# Autodesk Inventor assembly: chaimber
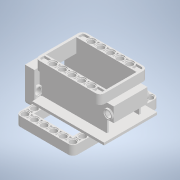
[picture p0: Inventor's stored thumbnail of the model, 180x180]
Saved by Autodesk Inventor 2021 (Build 250183000, 183)
## iProperties
Created: 2024-03-18
Part Number: chaimber
Document SubType Name: Assembly
Designer: 22hamfri
Author: 22hamfri
## Documents named in this file (5)
- C:\Users\22hamfri\Documents\School\Programmering\domino-bil\CAD\chaimber.iam
- C:\Users\22hamfri\Documents\School\Programmering\domino-bil\CAD\chaimber.ipt
- C:\Users\22hamfri\Documents\School\Programmering\domino-bil\CAD\chaimber-adapter.ipt
- C:\Users\22hamfri\Documents\School\Programmering\domino-bil\CAD\vehicle-adapter.ipt
- C:\Users\22hamfri\Documents\School\Programmering\domino-bil\CAD\magazine-adapter.ipt
## Components (4 placed, 4 different names)
1. chaimber:1 — Rigid:1, Rigid:2, Rigid:3
2. chaimber-adapter:1 — Rigid:2
3. vehicle-adapter:1 — Rigid:3
4. magazine-adapter:1 — Rigid:1
## Relationships (3: WeldJoint 3)
- Rigid:1 [WeldJoint]: chaimber:1 ↔ magazine-adapter:1
- Rigid:2 [WeldJoint]: chaimber:1 ↔ chaimber-adapter:1
- Rigid:3 [WeldJoint]: chaimber:1 ↔ vehicle-adapter:1
